# Autodesk Inventor assembly: mould_top_p1
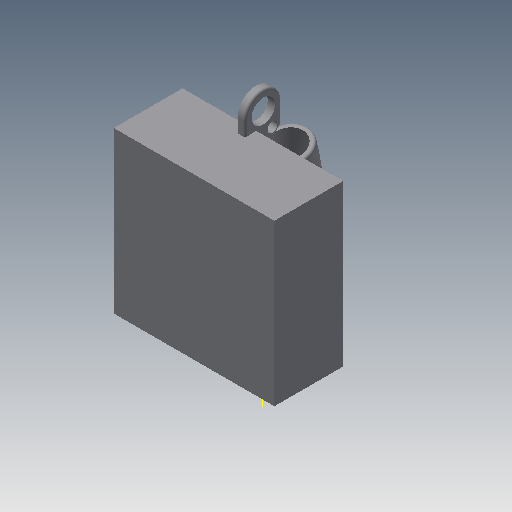
[picture p0: Inventor's stored thumbnail of the model, 512x512]
Saved by Autodesk Inventor 2017 (Build 210142000, 142)
## iProperties
Created: 2018-06-07
Part Number: mould_top_p1
Document SubType Name: Assembly
Designer: Nic
Author: Nic
## Documents named in this file (3)
- C:\Users\Nic\Documents\Antenna\mould_top_p1.iam
- C:\Users\Nic\Documents\Antenna\mould_casing.ipt
- C:\Users\Nic\Documents\Antenna\middle_segment_v2.ipt
## Components (2 placed, 2 different names)
1. mould_casing:1 — Insert:1
2. middle_segment_v2:1 — Insert:1
## Relationships (1: Insert 1)
- Insert:1: mould_casing:1 ↔ middle_segment_v2:1
